# Autodesk Inventor assembly: 1U_Satellite
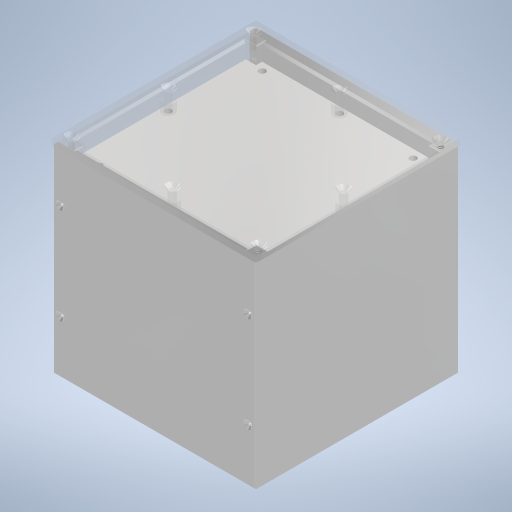
[picture p0: Inventor's stored thumbnail of the model, 512x512]
Saved by Autodesk Inventor 2023 (Build 270158000, 158)
## iProperties
Created: 2022-08-04
Part Number: 1U_Satellite
Document SubType Name: Assembly
Designer: Aditya Bansal
Mass: 656.857 g
Surface Area: 1290.28 cm^2
Volume: 243.28 cm^3
Density: 2.7 g/cm^3
Author: Aditya Bansal
## Documents named in this file (9)
- C:\Users\Aditya Bansal\OneDrive - UNSW\Uni\BlueSat\rocketry-datasat\Structure\V2\1U_Satellite.iam
- C:\Users\Aditya Bansal\OneDrive - UNSW\Uni\BlueSat\rocketry-datasat\Structure\V2\BottomPanel.ipt
- C:\Users\Aditya Bansal\OneDrive - UNSW\Uni\BlueSat\rocketry-datasat\Structure\V2\LeftPanel.ipt
- C:\Users\Aditya Bansal\OneDrive - UNSW\Uni\BlueSat\rocketry-datasat\Structure\V2\TopPanel.ipt
- C:\Users\Aditya Bansal\OneDrive - UNSW\Uni\BlueSat\rocketry-datasat\Structure\V2\FrontPanel.ipt
- C:\Users\Aditya Bansal\OneDrive - UNSW\Uni\BlueSat\rocketry-datasat\Structure\V2\RightPanel.ipt
- C:\Users\Aditya Bansal\OneDrive - UNSW\Uni\BlueSat\rocketry-datasat\Structure\V2\BackPanel.ipt
- C:\Users\Aditya Bansal\OneDrive - UNSW\Uni\BlueSat\rocketry-datasat\Structure\Electronics_Structure\ElectronicsBay.iam
- C:\Users\Aditya Bansal\OneDrive - UNSW\Uni\BlueSat\rocketry-datasat\Structure\Electronics_Structure\ElectronicsBayUpper.iam
## Components (8 placed, 8 different names)
1. BottomPanel:1 — Flush:1, Mate:1, Mate:2, Mate:3, Mate:11, Mate:12, Mate:16, Mate:17, Mate:18, Mate:19, Mate:20, Mate:21, Mate:22
2. LeftPanel:1 — Mate:8, Mate:9, Mate:11, Mate:12, Mate:13, Mate:14, Mate:15
3. TopPanel:1 — Mate:8, Mate:9, Mate:13, Mate:23, Mate:24
4. FrontPanel:1 — Mate:14, Mate:15
5. RightPanel:1 — Mate:16, Mate:17
6. BackPanel:1 — Mate:18, Mate:19
7. ElectronicsBay:1 [sub-assembly] — Mate:20, Mate:21, Mate:22
8. ElectronicsBayUpper:1 [sub-assembly] — Mate:23, Mate:24
## Relationships (20: Mate 19, Flush 1)
- Flush:1: BottomPanel:1
- Mate:1: BottomPanel:1
- Mate:2: BottomPanel:1
- Mate:3: BottomPanel:1
- Mate:8: LeftPanel:1 ↔ TopPanel:1
- Mate:9: LeftPanel:1 ↔ TopPanel:1
- Mate:11: BottomPanel:1 ↔ LeftPanel:1
- Mate:12: BottomPanel:1 ↔ LeftPanel:1
- Mate:13: LeftPanel:1 ↔ TopPanel:1
- Mate:14: LeftPanel:1 ↔ FrontPanel:1
- Mate:15: LeftPanel:1 ↔ FrontPanel:1
- Mate:16: BottomPanel:1 ↔ RightPanel:1
- Mate:17: BottomPanel:1 ↔ RightPanel:1
- Mate:18: BottomPanel:1 ↔ BackPanel:1
- Mate:19: BottomPanel:1 ↔ BackPanel:1
- Mate:20: BottomPanel:1 ↔ ElectronicsBay:1
- Mate:21: BottomPanel:1 ↔ ElectronicsBay:1
- Mate:22: BottomPanel:1 ↔ ElectronicsBay:1
- Mate:23: TopPanel:1 ↔ ElectronicsBayUpper:1
- Mate:24: TopPanel:1 ↔ ElectronicsBayUpper:1
